# Autodesk Inventor assembly: Contenedor Ensamblado
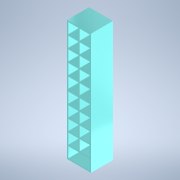
[picture p0: Inventor's stored thumbnail of the model, 180x180]
Saved by Autodesk Inventor 2020.3 (Build 243373000, 373)
## iProperties
Created: 2020-07-23
Part Number: Contenedor Ensamblado
Document SubType Name: Assembly
Designer: juanp
Author: juanp
## Documents named in this file (9)
- C:\Users\juanp\Desktop\ROBOCOL\Idea Final NAF\Contenedor Ensamblado.iam
- C:\Users\juanp\Desktop\ROBOCOL\Idea Final NAF\Contenedor A.ipt
- C:\Users\juanp\Desktop\ROBOCOL\Idea Final NAF\Contenedor B.ipt
- C:\Users\juanp\Desktop\ROBOCOL\Idea Final NAF\Contenedor Ensamblado\AIP\FEA\db7uk5ozk.fins
- C:\Users\juanp\Desktop\ROBOCOL\Idea Final NAF\Contenedor Ensamblado\AIP\FEA\db7uk5ozk.fsat
- C:\Users\juanp\Desktop\ROBOCOL\Idea Final NAF\Contenedor Ensamblado\AIP\FEA\db7uk5ozk.ftes
- C:\Users\juanp\Desktop\ROBOCOL\Idea Final NAF\Contenedor Ensamblado\AIP\FEA\db7uk5ozk.fwiz
- C:\Users\juanp\Desktop\ROBOCOL\Idea Final NAF\Contenedor Ensamblado\AIP\FEA\db7uk5p0g.fmsh
- C:\Users\juanp\Desktop\ROBOCOL\Idea Final NAF\Contenedor Ensamblado\AIP\FEA\db7uk5p0h.fres
## Components (2 placed, 2 different names)
1. Contenedor A:1 — Flush:2, Mate:1, Flush:3
2. Contenedor B:1 — Flush:2, Mate:1, Flush:3
## Relationships (3: Flush 2, Mate 1)
- Flush:2: Contenedor A:1 ↔ Contenedor B:1
- Mate:1: Contenedor A:1 ↔ Contenedor B:1
- Flush:3: Contenedor A:1 ↔ Contenedor B:1
